# Autodesk Inventor assembly: Celda_Robotizada_V1
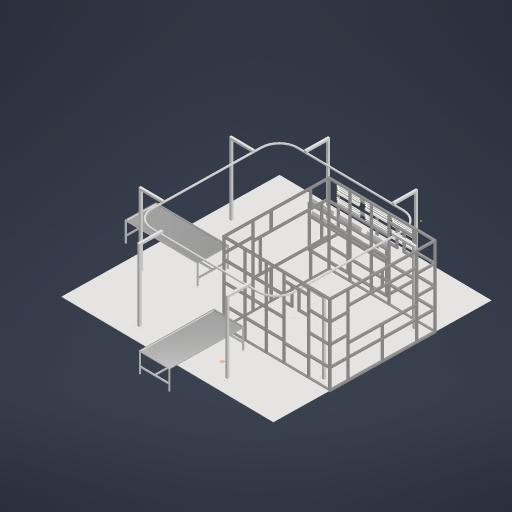
[picture p0: Inventor's stored thumbnail of the model, 512x512]
Saved by Autodesk Inventor 2024 (Build 280153000, 153)
## iProperties
Created: 2023-04-22
Part Number: Celda_Robotizada_V1
Document SubType Name: Assembly
Designer: javie
_SolveAssemblyDoc: Frame Generator Solve Assembly
_Version: 15.0.0
Author: javie
## Documents named in this file (11)
- C:\Users\javie\Downloads\Piezas CMR\Celda_Robotizada_V1.iam
- D:\Ensamble Celda Robotizada\Celda de Manufactura\Piso.ipt
- D:\Ensamble Celda Robotizada\Celda de Manufactura\IRB52.iam
- D:\Ensamble Celda Robotizada\Celda de Manufactura\Trs_Aereo.iam
- D:\Ensamble Celda Robotizada\Celda de Manufactura\GeoReferencia.ipt
- D:\Ensamble Celda Robotizada\Celda de Manufactura\Frame\Frame 1682207302696.iam
- D:\Ensamble Celda Robotizada\Celda de Manufactura\Gref_Sec.ipt
- D:\Ensamble Celda Robotizada\Celda de Manufactura\LamparaSe.iam
- D:\Ensamble Celda Robotizada\Celda de Manufactura\Mesa.ipt
- D:\Ensamble Celda Robotizada\Celda de Manufactura\str_mesa.ipt
- D:\Ensamble Celda Robotizada\Celda de Manufactura\Mesas.ipt
## Components (13 placed, 10 different names)
1. Piso:1 — Rígido:1, Rígido:2, Nivelación:1, Nivelación:2, Nivelación:3, Nivelación:4, Nivelación:5
2. IRB52:1 [sub-assembly] — Rígido:1
3. Trs_Aereo:1 [sub-assembly] — Rígido:2
4. GeoReferencia:1 — Nivelación:1
5. Frame 1682207302696:1 [sub-assembly] — Insertar:1, Insertar:2, Insertar:3
6. Gref_Sec:1 — Nivelación:2, Nivelación:3
7. LamparaSe:1 [sub-assembly] — Insertar:1
8. LamparaSe:2 [sub-assembly] — Insertar:2
9. LamparaSe:3 [sub-assembly] — Insertar:3
10. Mesa:1 — Nivelación:4, Nivelación:6, Rígido:3, Rígido:4
11. str_mesa:1 — Nivelación:5, Nivelación:6
12. Mesas:1 — Rígido:3
13. Mesas:2 — Rígido:4
## Relationships (13: Flush 6, WeldJoint 4, Insert 3)
- Rígido:1 [WeldJoint]: Piso:1 ↔ IRB52:1
- Rígido:2 [WeldJoint]: Piso:1 ↔ Trs_Aereo:1
- Nivelación:1 [Flush]: Piso:1 ↔ GeoReferencia:1
- Nivelación:2 [Flush]: Piso:1 ↔ Gref_Sec:1
- Nivelación:3 [Flush]: Piso:1 ↔ Gref_Sec:1
- Insertar:1: Frame 1682207302696:1 ↔ LamparaSe:1
- Insertar:2: Frame 1682207302696:1 ↔ LamparaSe:2
- Insertar:3: Frame 1682207302696:1 ↔ LamparaSe:3
- Nivelación:4 [Flush]: Piso:1 ↔ Mesa:1
- Nivelación:5 [Flush]: Piso:1 ↔ str_mesa:1
- Nivelación:6 [Flush]: Mesa:1 ↔ str_mesa:1
- Rígido:3 [WeldJoint]: Mesa:1 ↔ Mesas:1
- Rígido:4 [WeldJoint]: Mesa:1 ↔ Mesas:2
